# Autodesk Inventor assembly: Main_Assy
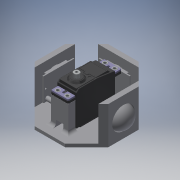
[picture p0: Inventor's stored thumbnail of the model, 180x180]
Saved by Autodesk Inventor 2017 (Build 210142000, 142)
## iProperties
Created: 2018-02-28
Part Number: Main_Assy
Document SubType Name: Assembly
Designer: Mitch
Author: Mitch
## Documents named in this file (4)
- E:\Youtube Channel\Pojects\Raspberry pi\PIR Camera\Main_Assy.iam
- E:\Youtube Channel\Pojects\Raspberry pi\PIR Camera\Main_assy_base.ipt
- E:\Youtube Channel\Pojects\Raspberry pi\PIR Camera\Servo Futaba S3003.ipt
- E:\Youtube Channel\Pojects\Raspberry pi\PIR Camera\PIR_Sensor.ipt
## Components (5 placed, 3 different names)
1. Main_assy_base:1 — Mate:2, Mate:3, Mate:4, Flush:3, Flush:4, Flush:5, Mate:5, Mate:6, Mate:7, Flush:6, Flush:7, Mate:8
2. Servo Futaba S3003:1 — Flush:6, Flush:7, Mate:8
3. PIR_Sensor:1 — Mate:2, Flush:4, Mate:6
4. PIR_Sensor:2 — Mate:4, Flush:5, Mate:7
5. PIR_Sensor:3 — Mate:3, Flush:3, Mate:5
## Relationships (12: Mate 7, Flush 5)
- Mate:2 (3.175 mm): Main_assy_base:1 ↔ PIR_Sensor:1
- Mate:3 (3.175 mm): Main_assy_base:1 ↔ PIR_Sensor:3
- Mate:4 (3.175 mm): Main_assy_base:1 ↔ PIR_Sensor:2
- Flush:3 (22.098 mm): Main_assy_base:1 ↔ PIR_Sensor:3
- Flush:4 (22.098 mm): Main_assy_base:1 ↔ PIR_Sensor:1
- Flush:5 (22.098 mm): Main_assy_base:1 ↔ PIR_Sensor:2
- Mate:5: Main_assy_base:1 ↔ PIR_Sensor:3
- Mate:6: Main_assy_base:1 ↔ PIR_Sensor:1
- Mate:7: Main_assy_base:1 ↔ PIR_Sensor:2
- Flush:6 (17.9578 mm): Main_assy_base:1 ↔ Servo Futaba S3003:1
- Flush:7 (28.4988 mm): Main_assy_base:1 ↔ Servo Futaba S3003:1
- Mate:8: Main_assy_base:1 ↔ Servo Futaba S3003:1
